# Autodesk Inventor assembly: Toughbox+Nano+All+Shafts+v2
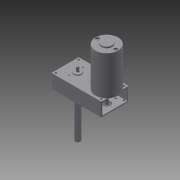
[picture p0: Inventor's stored thumbnail of the model, 180x180]
Saved by Autodesk Inventor 2015 (Build 190159000, 159)
## iProperties
Created: 2016-01-10
Part Number: Toughbox+Nano+All+Shafts+v2
Document SubType Name: Assembly
Designer: Applefamily
Title: Toughbox Nano All Shafts.STEP
Description: STEP AP203
Creation Date: 2015-02-02
Sending System: SolidWorks 2014
Preprocessor: SwSTEP 2.0
Author: Applefamily
## Documents named in this file (5)
- C:\Users\Applegate\Desktop\Chassy Files\Assembly\Imported Components\Toughbox+Nano+All+Shafts+v2\Toughbox+Nano+All+Shafts+v2.iam
- C:\Users\Applegate\Desktop\Chassy Files\Assembly\Imported Components\Toughbox+Nano+All+Shafts+v2\Toughbox Nano no Output Shaft.iam
- C:\Users\Applegate\Desktop\Chassy Files\Assembly\Imported Components\Toughbox+Nano+All+Shafts+v2\500-e-klip_smart.ipt
- C:\Users\Applegate\Desktop\Chassy Files\Assembly\Imported Components\Toughbox+Nano+All+Shafts+v2\CIM motor-1.ipt
- C:\Users\Applegate\Desktop\Chassy Files\Assembly\Imported Components\Toughbox+Nano+All+Shafts+v2\TB Output Shaft Hex Long.ipt
## Components (4 placed, 4 different names)
1. Toughbox Nano no Output Shaft_1 [sub-assembly] — Cylindrical:1, Flush:1
2. 500-e-klip_smart_2
3. CIM motor-1_4
4. TB Output Shaft Hex Long_5 — Cylindrical:1, Flush:1
## Relationships (2: CylindricalJoint 1, Flush 1)
- Cylindrical:1: Toughbox Nano no Output Shaft_1 ↔ TB Output Shaft Hex Long_5
- Flush:1 (-0.0508 mm): Toughbox Nano no Output Shaft_1 ↔ TB Output Shaft Hex Long_5
